# Autodesk Inventor assembly: Puzzle Cube Assembly
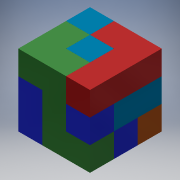
[picture p0: Inventor's stored thumbnail of the model, 180x180]
Saved by Autodesk Inventor 2018 (Build 220112000, 112)
## iProperties
Created: 2017-11-15
Part Number: Puzzle Cube Assembly
Document SubType Name: Assembly
Designer: 232963
Author: 232963
## Documents named in this file (6)
- P:\IED\Puzzle Cube\Puzzle Cube Assembly.iam
- P:\IED\Puzzle Cube\Red Part.ipt
- P:\IED\Puzzle Cube\Orange Part.ipt
- P:\IED\Puzzle Cube\Light Blue Part.ipt
- P:\IED\Puzzle Cube\Dark Blue Part.ipt
- P:\IED\Puzzle Cube\Green_Part.ipt
## Components (5 placed, 5 different names)
1. Red Part:1 — Rigid:3
2. Orange Part:1 — Rigid:1, Rigid:3
3. Light Blue Part:1 — Rigid:2
4. Green_Part:1 — Rigid:4
5. Dark Blue Part:1 — Rigid:1, Rigid:2, Rigid:4
## Relationships (4: WeldJoint 4)
- Rigid:1 [WeldJoint]: Orange Part:1 ↔ Dark Blue Part:1
- Rigid:2 [WeldJoint]: Light Blue Part:1 ↔ Dark Blue Part:1
- Rigid:3 [WeldJoint]: Red Part:1 ↔ Orange Part:1
- Rigid:4 [WeldJoint]: Green_Part:1 ↔ Dark Blue Part:1
